# Autodesk Inventor assembly: Elevator Sprocket with Sprockets_MIR2
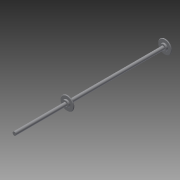
[picture p0: Inventor's stored thumbnail of the model, 180x180]
Saved by Autodesk Inventor 2015 (Build 190159000, 159)
## iProperties
Created: 2015-01-17
Part Number: Elevator Sprocket with Sprockets_MIR2
Document SubType Name: Assembly
Designer: chapale16
Author: chapale16
## Documents named in this file (3)
- H:\Elevator Sprocket with Sprockets_MIR2.iam
- H:\Elevator Axle_MIR3.ipt
- H:\Sprocket Large_MIR2.ipt
## Components (3 placed, 2 different names)
1. Elevator Axle_MIR3:1 — Mate:2
2. Sprocket Large_MIR2:1 — Flush:2
3. Sprocket Large_MIR2:2 — Mate:2, Flush:2
## Relationships (2: Mate 1, Flush 1)
- Mate:2: Elevator Axle_MIR3:1 ↔ Sprocket Large_MIR2:2
- Flush:2 (361.95 mm): Sprocket Large_MIR2:1 ↔ Sprocket Large_MIR2:2
